# Autodesk Inventor assembly: Wheel Assembly
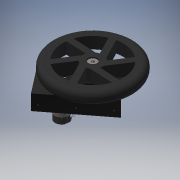
[picture p0: Inventor's stored thumbnail of the model, 180x180]
Saved by Autodesk Inventor 2017 (Build 210142000, 142)
## iProperties
Created: 2018-10-18
Part Number: Wheel Assembly
Document SubType Name: Assembly
Designer: Dell
Author: Dell
## Documents named in this file (7)
- C:\Users\Dell\Documents\GitHub\tr2\Wheel Assembly\Wheel Assembly, Left.iam
- C:\Users\Dell\Documents\GitHub\tr2\Wheel Assembly\Scooter Wheel.ipt
- C:\Users\Dell\Documents\GitHub\tr2\Wheel Assembly\Wheel Assembly\Design Accelerator\Spur Gears1.iam
- C:\Users\Dell\Documents\GitHub\tr2\Base\37d-gearmotor-50-70-encoder.ipt
- C:\Users\Dell\Documents\GitHub\tr2\Wheel Assembly\22x8x8mm Bearing.ipt
- C:\Users\Dell\Documents\GitHub\tr2\Wheel Assembly\6mm Mounting Hub, thin.ipt
- C:\Users\Dell\Documents\GitHub\tr2\Wheel Assembly\WA02.ipt
## Components (12 placed, 6 different names)
1. WA02:1 — Mate:51, Mate:52, Mate:53, Mate:54, Mate:55, Mate:56, Mate:57, Mate:59, Mate:60
2. Scooter Wheel:1 — Mate:25, Mate:26, Mate:27, Mate:28, Mate:47, Rotation:1
3. Spur Gears:1 [sub-assembly] — Mate:21, Mate:22, Mate:45, Mate:47, Rotation:1, Mate:48, Mate:49, Mate:50, Mate:52, Mate:60
4. 37d-gearmotor-50-70-encoder:1 — Mate:20, Mate:45, Mate:53, Mate:54
5. 22x8x8mm Bearing:1 — Mate:37, Mate:48
6. 22x8x8mm Bearing:2 — Mate:37, Mate:49, Mate:57, Mate:58
7. 6mm Mounting Hub, thin:1 — Mate:20, Mate:21, Mate:22
8. 22x8x8mm Bearing:3 — Mate:34, Mate:41, Mate:51, Mate:55, Mate:56
9. 22x8x8mm Bearing:4 — Mate:25, Mate:26
10. 22x8x8mm Bearing:5 — Mate:27, Mate:28, Mate:34, Mate:50
11. 22x8x8mm Bearing:6 — Mate:41
12. 22x8x8mm Bearing:7 — Mate:58, Mate:59
## Relationships (26: Mate 25, RelateRotation 1)
- Mate:20: 37d-gearmotor-50-70-encoder:1 ↔ 6mm Mounting Hub, thin:1
- Mate:21: Spur Gears:1 ↔ 6mm Mounting Hub, thin:1
- Mate:22: Spur Gears:1 ↔ 6mm Mounting Hub, thin:1
- Mate:25: Scooter Wheel:1 ↔ 22x8x8mm Bearing:4
- Mate:26: Scooter Wheel:1 ↔ 22x8x8mm Bearing:4
- Mate:27: Scooter Wheel:1 ↔ 22x8x8mm Bearing:5
- Mate:28: Scooter Wheel:1 ↔ 22x8x8mm Bearing:5
- Mate:34: 22x8x8mm Bearing:3 ↔ 22x8x8mm Bearing:5
- Mate:37: 22x8x8mm Bearing:1 ↔ 22x8x8mm Bearing:2
- Mate:41: 22x8x8mm Bearing:3 ↔ 22x8x8mm Bearing:6
- Mate:45: Spur Gears:1 ↔ 37d-gearmotor-50-70-encoder:1
- Mate:47: Scooter Wheel:1 ↔ Spur Gears:1
- Rotation:1 [RelateRotation] (1 ul): Scooter Wheel:1 ↔ Spur Gears:1
- Mate:48: Spur Gears:1 ↔ 22x8x8mm Bearing:1
- Mate:49: Spur Gears:1 ↔ 22x8x8mm Bearing:2
- Mate:50: Spur Gears:1 ↔ 22x8x8mm Bearing:5
- Mate:51: WA02:1 ↔ 22x8x8mm Bearing:3
- Mate:52: WA02:1 ↔ Spur Gears:1
- Mate:53: WA02:1 ↔ 37d-gearmotor-50-70-encoder:1
- Mate:54: WA02:1 ↔ 37d-gearmotor-50-70-encoder:1
- Mate:55: WA02:1 ↔ 22x8x8mm Bearing:3
- Mate:56: WA02:1 ↔ 22x8x8mm Bearing:3
- Mate:57: WA02:1 ↔ 22x8x8mm Bearing:2
- Mate:58: 22x8x8mm Bearing:2 ↔ 22x8x8mm Bearing:7
- Mate:59: WA02:1 ↔ 22x8x8mm Bearing:7
- Mate:60: WA02:1 ↔ Spur Gears:1
